# Autodesk Inventor assembly: Snap-Twist Assembly
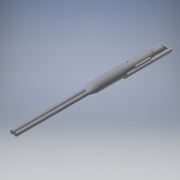
[picture p0: Inventor's stored thumbnail of the model, 180x180]
Saved by Autodesk Inventor 2016 (Build 200138000, 138)
## iProperties
Created: 2015-08-07
Part Number: Snap-Twist Assembly
Document SubType Name: Assembly
Designer: Nancy
Mass: 0.301267 g
Surface Area: 6.79617 cm^2
Volume: 0.301267 cm^3
Density: 1 g/cm^3
Author: Nancy
## Documents named in this file (3)
- C:\Users\Nancy\Documents\Inventor\mXers Technologies\Snap-Twist Assembly.iam
- C:\Users\Nancy\Documents\Inventor\mXers Technologies\Snap-Twist Idea F.ipt
- C:\Users\Nancy\Documents\Inventor\mXers Technologies\Snap-Twist Idea M.ipt
## Components (2 placed, 2 different names)
1. Snap-Twist Idea F:1 — Insert:1
2. Snap-Twist Idea M:1 — Insert:1
## Relationships (1: Insert 1)
- Insert:1 (-15.0114 mm): Snap-Twist Idea F:1 ↔ Snap-Twist Idea M:1
